# Autodesk Inventor assembly: jst 1
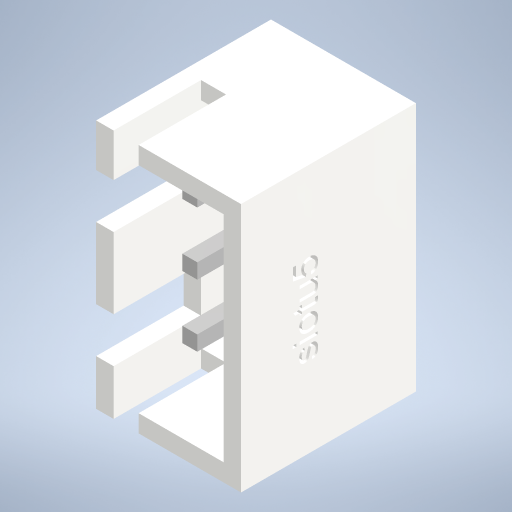
[picture p0: Inventor's stored thumbnail of the model, 512x512]
Saved by Autodesk Inventor 2024 (Build 280153000, 153)
## iProperties
Created: 2023-09-07
Part Number: jst 1
Document SubType Name: Assembly
Designer: Roman Suk
Sending System: Autodesk Translation Framework v12.9.0.99
Preprocessor: ST-DEVELOPER v20
Title: jst 1 v4.step
## Documents named in this file (3)
- C:\Users\Roman Suk\Documents\Ročníkovka SŠ\Technical documentation\Final\jst 1 v4\jst 1 v4.iam
- C:\Users\Roman Suk\Documents\Ročníkovka SŠ\Technical documentation\Final\jst 1 v4\Bileşen1.ipt
- C:\Users\Roman Suk\Documents\Ročníkovka SŠ\Technical documentation\Final\jst 1 v4\Bileşen2.ipt
## Components (4 placed, 2 different names)
1. Bileşen1:1 — Flush:1, Flush:2, Mate:1, Mate:2, Mate:3, Mate:4
2. Bileşen2:1
3. Bileşen2:2 — Flush:1, Mate:1, Mate:2
4. Bileşen2:3 — Flush:2, Mate:3, Mate:4
## Relationships (6: Mate 4, Flush 2)
- Flush:1: Bileşen1:1 ↔ Bileşen2:2
- Flush:2: Bileşen1:1 ↔ Bileşen2:3
- Mate:1: Bileşen1:1 ↔ Bileşen2:2
- Mate:2: Bileşen1:1 ↔ Bileşen2:2
- Mate:3: Bileşen1:1 ↔ Bileşen2:3
- Mate:4: Bileşen1:1 ↔ Bileşen2:3
